# Autodesk Inventor assembly: forearm_block
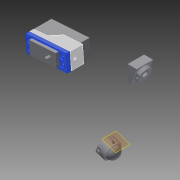
[picture p0: Inventor's stored thumbnail of the model, 180x180]
Saved by Autodesk Inventor 2015 (Build 190159000, 159)
## iProperties
Created: 2015-09-26
Part Number: forearm_block
Document SubType Name: Assembly
Designer: astralien3000
Author: astralien3000
## Documents named in this file (8)
- C:\Users\astralien3000\Desktop\buggybot2\meca\v2016\forearm_block.iam
- C:\Users\astralien3000\Desktop\buggybot2\meca\v2016\optoforce_base.ipt
- C:\Users\astralien3000\Desktop\buggybot2\meca\lib\optoforce.ipt
- C:\Users\astralien3000\Desktop\buggybot2\meca\lib\servo.ipt
- C:\Users\astralien3000\Desktop\buggybot2\meca\v2016\forearm_anti_axe.ipt
- C:\Users\astralien3000\Desktop\buggybot2\meca\v2016\forearm_1.ipt
- C:\Users\astralien3000\Desktop\buggybot2\meca\v2016\forearm_2.ipt
- C:\Users\astralien3000\Desktop\buggybot2\meca\v2016\forearm_3.ipt
## Components (7 placed, 7 different names)
1. optoforce_base:1 — Placage:5, Placage:6
2. optoforce:1 — Placage:5, Placage:6
3. servo:1 — Placage:14, Placage:18, Placage:19
4. forearm_anti_axe:1 — Placage:15, Placage:16, Placage:17
5. forearm_1:1 — Placage:10, Placage:11, Placage:12, Placage:14, Placage:15, Placage:16, Placage:17, Placage:18, Placage:19
6. forearm_2:1 — Placage:10, Placage:11, Placage:12
7. forearm_3:1
## Relationships (11: Mate 11)
- Placage:5 [Mate]: optoforce_base:1 ↔ optoforce:1
- Placage:6 [Mate]: optoforce_base:1 ↔ optoforce:1
- Placage:10 [Mate]: forearm_1:1 ↔ forearm_2:1
- Placage:11 [Mate]: forearm_1:1 ↔ forearm_2:1
- Placage:12 [Mate]: forearm_1:1 ↔ forearm_2:1
- Placage:14 [Mate]: servo:1 ↔ forearm_1:1
- Placage:15 [Mate]: forearm_anti_axe:1 ↔ forearm_1:1
- Placage:16 [Mate]: forearm_anti_axe:1 ↔ forearm_1:1
- Placage:17 [Mate]: forearm_anti_axe:1 ↔ forearm_1:1
- Placage:18 [Mate] (0.5 mm): servo:1 ↔ forearm_1:1
- Placage:19 [Mate] (0.5 mm): servo:1 ↔ forearm_1:1
